# Autodesk Inventor assembly: Handlling Module
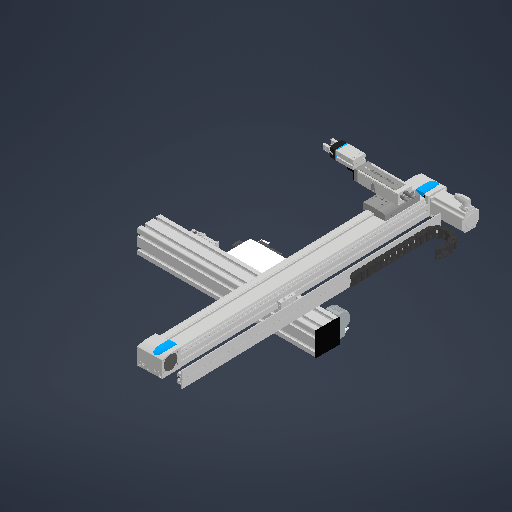
[picture p0: Inventor's stored thumbnail of the model, 512x512]
Saved by Autodesk Inventor 2027 (Build 310192000, 192)
## iProperties
Created: 2026-04-25
Part Number: Handlling Module
Document SubType Name: Assembly
Designer: ratik
Author: ratik
## Documents named in this file (14)
- C:\Users\ratik\OneDrive\Personal Folder\00_Startup\01_Mectosys_Prototype\01_Prototype\01_Mechanical\3D file\Assembly File\Handlling Module.iam
- C:\Users\ratik\OneDrive\Personal Folder\00_Startup\01_Mectosys_Prototype\01_Prototype\01_Mechanical\3D file\06_Handlling Station\03_EGC-80-700-TB-KF-0H-GK  Belt axis\AIS2024\556814 EGC-80-700-TB-KF-0H-GK_(0).iam
- C:\Users\ratik\OneDrive\Personal Folder\00_Startup\01_Mectosys_Prototype\01_Prototype\01_Mechanical\3D file\06_Handlling Station\01_EMMS-ST-57-M-SE-G2 Motor\8156180 EMMT-ST-57-L-RS---(400).ipt
- C:\Users\ratik\OneDrive\Personal Folder\00_Startup\01_Mectosys_Prototype\01_Prototype\01_Mechanical\3D file\06_Handlling Station\05_DGSL-12-50-Y3A Cylinder\AIS2024\543979 DGSL-12-50-Y3A---(0).iam
- C:\Users\ratik\OneDrive\Personal Folder\00_Startup\01_Mectosys_Prototype\01_Prototype\01_Mechanical\3D file\06_Handlling Station\06_DHRS-25-A Gripper\AIS2024\1310162 DHRS-25-A---(0).iam
- C:\Users\ratik\OneDrive\Personal Folder\00_Startup\01_Mectosys_Prototype\01_Prototype\01_Mechanical\3D file\06_Handlling Station\cable-drag-chain-10x20mm-1.snapshot.1\Drag Chain 10x20\Drag Chain 10x20.ipt
- C:\Users\ratik\OneDrive\Personal Folder\00_Startup\01_Mectosys_Prototype\01_Prototype\01_Mechanical\3D file\06_Handlling Station\Mounting bracket\AIS2024\558043 MUE-70_80---(70).iam
- C:\Users\ratik\OneDrive\Personal Folder\00_Startup\01_Mectosys_Prototype\01_Prototype\01_Mechanical\3D file\06_Handlling Station\HFS8-8080-1000_Inventor\HFS8-8080-1000.ipt
- C:\Users\ratik\OneDrive\Personal Folder\00_Startup\01_Mectosys_Prototype\01_Prototype\01_Mechanical\3D file\06_Handlling Station\End cap\HFC8-8080-B.ipt
- C:\Users\ratik\OneDrive\Personal Folder\00_Startup\01_Mectosys_Prototype\01_Prototype\01_Mechanical\3D file\06_Handlling Station\Cylinder holding bracket.ipt
- C:\Users\ratik\OneDrive\Personal Folder\00_Startup\01_Mectosys_Prototype\01_Prototype\01_Mechanical\3D file\06_Handlling Station\02_CMMT-ST-C8-1C-PN-S0 Drive\AIS2024\8163946 CMMT-ST-C8-1C-MP-S0---(high).iam
- C:\Users\ratik\OneDrive\Personal Folder\00_Startup\01_Mectosys_Prototype\01_Prototype\01_Mechanical\3D file\02_Slider\09_HFSFIN6-1554-1000_STEP_AP214_20260415\HFSFIN6-1554-1000\HFSFIN6-1554-1000.ipt
- C:\Users\ratik\OneDrive\Personal Folder\00_Startup\01_Mectosys_Prototype\01_Prototype\01_Mechanical\3D file\06_Handlling Station\Valve\AIS2024\578162 VUVG-L10-M52-MT-M5-1H2L-W1.iam
- C:\Users\ratik\OneDrive\Personal Folder\00_Startup\01_Mectosys_Prototype\01_Prototype\01_Mechanical\3D file\03_Conveyor Assembly\23_181857052-9-2903801\2903801.ipt
## Components (15 placed, 13 different names)
1. 556814 EGC-80-700-TB-KF-0H-GK_(0):1 [sub-assembly] — Mate:2, Mate:3, Mate:5, Mate:6, Flush:6, Mate:11
2. 8156180 EMMT-ST-57-L-RS---(400):1 — Mate:2
3. 543979 DGSL-12-50-Y3A---(0):1 [sub-assembly] — Mate:3, Mate:8, Flush:4, Flush:5
4. 1310162 DHRS-25-A---(0):1 [sub-assembly] — Mate:9
5. Drag Chain 10x20:1 — Mate:12
6. 558043 MUE-70_80---(70):1 [sub-assembly] — Mate:5
7. HFS8-8080-1000:1 — Mate:6, Mate:7, Flush:1, Flush:2, Mate:10, Mate:13
8. HFC8-8080-B:1 — Mate:7, Flush:1, Flush:2
9. Cylinder holding bracket:1 — Mate:8, Flush:4, Flush:5, Mate:9
10. 8163946 CMMT-ST-C8-1C-MP-S0---(high):1 [sub-assembly] — Mate:10
11. HFSFIN6-1554-1000:1 — Flush:6, Mate:11, Mate:12
12. 578162 VUVG-L10-M52-MT-M5-1H2L-W1:1 [sub-assembly] — Mate:13, Mate:14, Mate:16
13. 578162 VUVG-L10-M52-MT-M5-1H2L-W1:2 [sub-assembly] — Mate:14, Mate:15, Mate:16, Mate:17
14. 578162 VUVG-L10-M52-MT-M5-1H2L-W1:3 [sub-assembly] — Mate:15, Mate:17
15. 2903801:1
## Relationships (20: Mate 15, Flush 5)
- Mate:2: 556814 EGC-80-700-TB-KF-0H-GK_(0):1 ↔ 8156180 EMMT-ST-57-L-RS---(400):1
- Mate:3: 556814 EGC-80-700-TB-KF-0H-GK_(0):1 ↔ 543979 DGSL-12-50-Y3A---(0):1
- Mate:5: 556814 EGC-80-700-TB-KF-0H-GK_(0):1 ↔ 558043 MUE-70_80---(70):1
- Mate:6: 556814 EGC-80-700-TB-KF-0H-GK_(0):1 ↔ HFS8-8080-1000:1
- Mate:7: HFS8-8080-1000:1 ↔ HFC8-8080-B:1
- Flush:1: HFS8-8080-1000:1 ↔ HFC8-8080-B:1
- Flush:2: HFS8-8080-1000:1 ↔ HFC8-8080-B:1
- Mate:8: 543979 DGSL-12-50-Y3A---(0):1 ↔ Cylinder holding bracket:1
- Flush:4: 543979 DGSL-12-50-Y3A---(0):1 ↔ Cylinder holding bracket:1
- Flush:5: 543979 DGSL-12-50-Y3A---(0):1 ↔ Cylinder holding bracket:1
- Mate:9: 1310162 DHRS-25-A---(0):1 ↔ Cylinder holding bracket:1
- Mate:10: HFS8-8080-1000:1 ↔ 8163946 CMMT-ST-C8-1C-MP-S0---(high):1
- Flush:6: 556814 EGC-80-700-TB-KF-0H-GK_(0):1 ↔ HFSFIN6-1554-1000:1
- Mate:11 (50 mm): 556814 EGC-80-700-TB-KF-0H-GK_(0):1 ↔ HFSFIN6-1554-1000:1
- Mate:12: Drag Chain 10x20:1 ↔ HFSFIN6-1554-1000:1
- Mate:13: HFS8-8080-1000:1 ↔ 578162 VUVG-L10-M52-MT-M5-1H2L-W1:1
- Mate:14: 578162 VUVG-L10-M52-MT-M5-1H2L-W1:1 ↔ 578162 VUVG-L10-M52-MT-M5-1H2L-W1:2
- Mate:15: 578162 VUVG-L10-M52-MT-M5-1H2L-W1:2 ↔ 578162 VUVG-L10-M52-MT-M5-1H2L-W1:3
- Mate:16: 578162 VUVG-L10-M52-MT-M5-1H2L-W1:1 ↔ 578162 VUVG-L10-M52-MT-M5-1H2L-W1:2
- Mate:17: 578162 VUVG-L10-M52-MT-M5-1H2L-W1:2 ↔ 578162 VUVG-L10-M52-MT-M5-1H2L-W1:3
